# Autodesk Inventor assembly: Assembly1
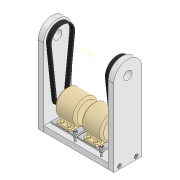
[picture p0: Inventor's stored thumbnail of the model, 180x180]
Saved by Autodesk Inventor 2022.5 (Build 265521000, 521)
## iProperties
Created: 2020-07-24
Part Number: Assembly1
Document SubType Name: Assembly
Designer: admin
Author: admin
## Documents named in this file (9)
- F:\YouTube\2024\YouTube\11N\9BevelGear2DoF\AssemblyFrame.iam
- F:\YouTube\2024\YouTube\11N\9BevelGear2DoF\Bearing.ipt
- F:\YouTube\2024\YouTube\11N\9BevelGear2DoF\Bottom.ipt
- F:\YouTube\2024\YouTube\11N\9BevelGear2DoF\Motor1x40.ipt
- F:\YouTube\2024\YouTube\11N\9BevelGear2DoF\Belt.ipt
- F:\YouTube\2024\YouTube\11N\9BevelGear2DoF\MotorBase.ipt
- F:\YouTube\2024\YouTube\11N\9BevelGear2DoF\PinScrew.ipt
- F:\YouTube\2024\YouTube\11N\9BevelGear2DoF\Nut3.ipt
- F:\YouTube\2024\YouTube\11N\9BevelGear2DoF\Bolt3G.ipt
## Components (25 placed, 8 different names)
1. Motor1x40:1 — Mate:19, Flush:4, Mate:25, Mate:31, Flush:6
2. Motor1x40:2 — Mate:21, Flush:4, Mate:32
3. Bearing:2 — Flush:2, Flush:3, Mate:16, Mate:21, Mate:33, Mate:39, Flush:12, Insert:12, Insert:13
4. Bottom:1 — Flush:2, Flush:3, Mate:16, Flush:5, Mate:40, Flush:11
5. Belt:1 — Mate:25, Mate:37, Mate:38
6. Belt:2 — Mate:37, Mate:38, Mate:39
7. MotorBase:1 — Mate:31, Flush:5, Flush:6, Flush:7, Mate:34, Insert:4, Insert:5, Mate:36, Insert:6, Insert:7
8. MotorBase:2 — Mate:32, Flush:7, Mate:33, Insert:1, Insert:2, Insert:3, Mate:35, Insert:8, Insert:9
9. PinScrew:1 — Insert:1, Flush:8
10. Nut3:1 — Insert:2
11. Nut3:2 — Insert:3
12. PinScrew:2 — Mate:35, Flush:10
13. Nut3:3 — Insert:6
14. Nut3:4 — Insert:7
15. PinScrew:3 — Mate:36, Flush:9
16. Nut3:5 — Insert:8
17. Nut3:6 — Insert:9
18. PinScrew:4 — Mate:34, Flush:8, Flush:9, Flush:10
19. Nut3:7 — Insert:4
20. Nut3:8 — Insert:5
21. Bearing:3 — Mate:40, Flush:11, Flush:12, Insert:10, Insert:11
22. Bolt3G:1 — Insert:10
23. Bolt3G:2 — Insert:11
24. Bolt3G:3 — Insert:13
25. Bolt3G:4 — Insert:12
## Relationships (38: Mate 14, Insert 13, Flush 11)
- Flush:2: Bearing:2 ↔ Bottom:1
- Flush:3: Bearing:2 ↔ Bottom:1
- Mate:16: Bearing:2 ↔ Bottom:1
- Mate:19: Motor1x40:1
- Mate:21 (12 mm): Motor1x40:2 ↔ Bearing:2
- Flush:4: Motor1x40:1 ↔ Motor1x40:2
- Mate:25: Motor1x40:1 ↔ Belt:1
- Mate:31: Motor1x40:1 ↔ MotorBase:1
- Flush:5: Bottom:1 ↔ MotorBase:1
- Flush:6 (2.5 mm): Motor1x40:1 ↔ MotorBase:1
- Mate:32: Motor1x40:2 ↔ MotorBase:2
- Flush:7: MotorBase:1 ↔ MotorBase:2
- Mate:33 (10 mm): Bearing:2 ↔ MotorBase:2
- Insert:1 (3 mm): MotorBase:2 ↔ PinScrew:1
- Insert:2: MotorBase:2 ↔ Nut3:1
- Insert:3: MotorBase:2 ↔ Nut3:2
- Mate:34: MotorBase:1 ↔ PinScrew:4
- Flush:8: PinScrew:1 ↔ PinScrew:4
- Insert:4: MotorBase:1 ↔ Nut3:7
- Insert:5: MotorBase:1 ↔ Nut3:8
- Mate:35: MotorBase:2 ↔ PinScrew:2
- Mate:36: MotorBase:1 ↔ PinScrew:3
- Flush:9: PinScrew:3 ↔ PinScrew:4
- Flush:10: PinScrew:2 ↔ PinScrew:4
- Insert:6: MotorBase:1 ↔ Nut3:3
- Insert:7: MotorBase:1 ↔ Nut3:4
- Insert:8: MotorBase:2 ↔ Nut3:5
- Insert:9: MotorBase:2 ↔ Nut3:6
- Mate:37: Belt:1 ↔ Belt:2
- Mate:38: Belt:1 ↔ Belt:2
- Mate:39 (1 mm): Bearing:2 ↔ Belt:2
- Mate:40: Bottom:1 ↔ Bearing:3
- Flush:11: Bottom:1 ↔ Bearing:3
- Flush:12: Bearing:2 ↔ Bearing:3
- Insert:10: Bearing:3 ↔ Bolt3G:1
- Insert:11: Bearing:3 ↔ Bolt3G:2
- Insert:12: Bearing:2 ↔ Bolt3G:4
- Insert:13: Bearing:2 ↔ Bolt3G:3
